# Autodesk Inventor assembly: A Drive Assembly
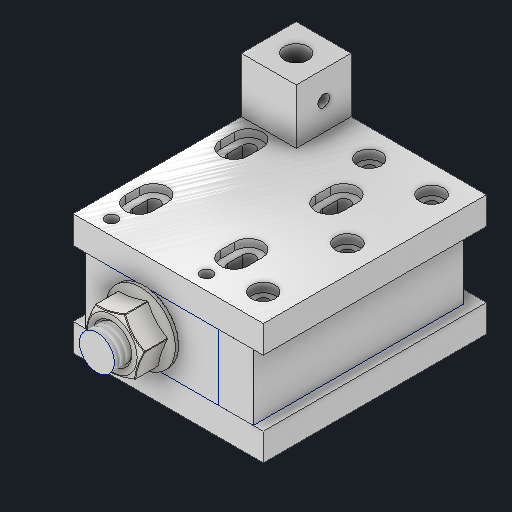
[picture p0: Inventor's stored thumbnail of the model, 512x512]
Saved by Autodesk Inventor 2025.1 (Build 291241020, 241B)
## iProperties
Created: 2025-04-19
Part Number: A Drive Assembly
Document SubType Name: Assembly
Designer: Joshua Eah
Mass: 449.057 g
Surface Area: 327.089 cm^2
Volume: 68.6532 cm^3
Density: 6.54094 g/cm^3
Author: Joshua Eah
## Documents named in this file (9)
- C:\Users\Joshua Eah\Documents\Voron 0.2\CAD\Machined Parts\AB Drives\A Drive\A Drive Assembly.iam
- C:\Users\Joshua Eah\Documents\Voron 0.2\CAD\Machined Parts\AB Drives\A Drive\A Drive Frame Lower.ipt
- C:\Users\Joshua Eah\Documents\Voron 0.2\CAD\Machined Parts\AB Drives\A Drive\A Drive Frame Upper.ipt
- C:\Users\Joshua Eah\Documents\Voron 0.2\CAD\Machined Parts\AB Drives\Drive Tensioner Rod\Tensioner Rod.ipt
- C:\Users\Joshua Eah\Documents\Voron 0.2\CAD\Machined Parts\AB Drives\Drive Tensioner\Drive Tensioner.ipt
- C:\Users\Joshua Eah\Documents\Voron 0.2\CAD\Machined Parts\AB Drives\Drive Frame Bearing Plate\Drive Frame Tension Bearing Plate.ipt
- C:\Users\Joshua Eah\Documents\Voron 0.2\CAD\Machined Parts\AB Drives\3_8_16_Nut.ipt
- C:\Users\Joshua Eah\Documents\Voron 0.2\CAD\Machined Parts\AB Drives\Drive Frame Spacer\Drive Frame Spacing Block.ipt
- C:\Users\Joshua Eah\Documents\Voron 0.2\CAD\Machined Parts\Spacers\Spacer.ipt
## Components (8 placed, 8 different names)
1. A Drive Frame Lower:1 — Slider:1, Insert:1, Insert:2, Insert:3
2. A Drive Frame Upper:1 — Insert:4, Mate:1
3. Drive Tensioner:1 — Rigid:1, Slider:1
4. Tensioner Rod:1 — Rigid:1, Cylindrical:1
5. Drive Frame Tension Bearing Plate:1 — Insert:1, Insert:2
6. 3_8_16_Nut:1 — Cylindrical:1
7. Drive Frame Spacing Block:1 — Insert:3, Insert:4
8. Spacer:1 — Mate:1
## Relationships (8: Insert 4, WeldJoint 1, TranslationJoint 1, CylindricalJoint 1, Mate 1)
- Rigid:1 [WeldJoint]: Drive Tensioner:1 ↔ Tensioner Rod:1
- Slider:1 [TranslationJoint]: A Drive Frame Lower:1 ↔ Drive Tensioner:1
- Cylindrical:1: Tensioner Rod:1 ↔ 3_8_16_Nut:1
- Insert:1: A Drive Frame Lower:1 ↔ Drive Frame Tension Bearing Plate:1
- Insert:2: A Drive Frame Lower:1 ↔ Drive Frame Tension Bearing Plate:1
- Insert:3: A Drive Frame Lower:1 ↔ Drive Frame Spacing Block:1
- Insert:4: A Drive Frame Upper:1 ↔ Drive Frame Spacing Block:1
- Mate:1: A Drive Frame Upper:1 ↔ Spacer:1
